# Autodesk Inventor assembly: driveFrameV2
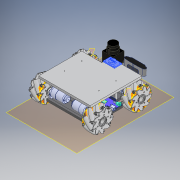
[picture p0: Inventor's stored thumbnail of the model, 180x180]
Saved by Autodesk Inventor 2017 (Build 210142000, 142)
## iProperties
Created: 2017-03-10
Part Number: driveFrameV2
Document SubType Name: Assembly
Designer: Naga
Author: Naga
## Documents named in this file (15)
- E:\GDrive\IEEE CS\SoutheastCon2017\Cad\Chassis\driveFrameV2.iam
- E:\GDrive\IEEE CS\SoutheastCon2017\Cad\Chassis\BottomPlateV2.ipt
- E:\GDrive\IEEE CS\SoutheastCon2017\Cad\Motors\37DEncoderAlBlock.iam
- E:\GDrive\IEEE CS\SoutheastCon2017\Cad\Chassis\TopPlateV1.ipt
- E:\GDrive\IEEE CS\SoutheastCon2017\Cad\Chassis\postSpacer.ipt
- E:\GDrive\IEEE CS\SoutheastCon2017\Cad\tilt\step\tiltservomount_std.iam
- E:\GDrive\IEEE CS\SoutheastCon2017\Cad\tilt\TiltMountShort.iam
- E:\GDrive\IEEE CS\SoutheastCon2017\Cad\pan\base.ipt
- E:\GDrive\IEEE CS\SoutheastCon2017\Cad\Motors\100mm Aluminum Mecanum wheels.iam
- E:\GDrive\IEEE CS\SoutheastCon2017\Cad\Electronics\Arduino Mega 2560.ipt
- E:\GDrive\IEEE CS\SoutheastCon2017\Cad\Electronics\RaspberryPi2 STEP214.iam
- E:\GDrive\IEEE CS\SoutheastCon2017\Cad\Electronics\kangarooSaberTooth.iam
- E:\GDrive\IEEE CS\SoutheastCon2017\Cad\Electronics\Lidar.ipt
- E:\GDrive\IEEE CS\SoutheastCon2017\Cad\Electronics\camera\LogitechC920Montaj.ipt
- E:\GDrive\IEEE CS\SoutheastCon2017\Cad\Motors\MG995_Servo.iam
## Components (24 placed, 14 different names)
1. BottomPlateV2:1 — Mate:3, Mate:4, Mate:5, Mate:6, Mate:7, Mate:8, Mate:9, Mate:16, Mate:20, Mate:21, Mate:22, Mate:23, Mate:24, Mate:25, Mate:26, Mate:50, Mate:51, Mate:52, Mate:53, Flush:26, Flush:27, Flush:29, Flush:30, Mate:56, Flush:33, Flush:38
2. 37DEncoderAlBlock:1 [sub-assembly] — Flush:2, Flush:3, Mate:5, Flush:4, Mate:6, Mate:48, Mate:49
3. 37DEncoderAlBlock:2 [sub-assembly] — Flush:1, Flush:5, Mate:9, Mate:44, Mate:46
4. 37DEncoderAlBlock:3 [sub-assembly] — Flush:3, Flush:5, Mate:8, Mate:45, Mate:47
5. 37DEncoderAlBlock:4 [sub-assembly] — Flush:1, Flush:2, Flush:4, Mate:7, Mate:42, Mate:43
6. TopPlateV1:1 — Mate:20, Mate:21, Mate:27, Mate:35, Flush:21, Mate:62
7. postSpacer:1 — Mate:24, Flush:12
8. postSpacer:2 — Mate:22, Flush:13, Flush:14, Mate:27
9. postSpacer:3 — Mate:23, Mate:26, Flush:12, Flush:13
10. postSpacer:4 — Mate:25, Flush:14
11. TiltMountShort:2 [sub-assembly] — Mate:31, Mate:56, Mate:57, Flush:33, Mate:59, Flush:38
12. tiltservomount_std:2 [sub-assembly] — Mate:31, Mate:55, Flush:31, Flush:32, Mate:57, Mate:60, Mate:61
13. base:1 — Mate:35, Flush:21
14. 100mm Aluminum Mecanum wheels:1 [sub-assembly] — Mate:42, Mate:43
15. 100mm Aluminum Mecanum wheels:2 [sub-assembly] — Mate:44, Mate:46
16. 100mm Aluminum Mecanum wheels:3 [sub-assembly] — Mate:45, Mate:47
17. 100mm Aluminum Mecanum wheels:4 [sub-assembly] — Mate:48, Mate:49
18. Arduino Mega 2560:1 — Mate:53, Flush:26
19. RaspberryPi2 STEP214:1 [sub-assembly] — Mate:52, Flush:27
20. kangarooSaberTooth:1 [sub-assembly] — Mate:51, Flush:29, Mate:54
21. kangarooSaberTooth:2 [sub-assembly] — Mate:50, Flush:30, Mate:54
22. Lidar:1 — Mate:55, Flush:31, Flush:32
23. LogitechC920Montaj:1 — Mate:62
24. MG995_Servo:1 [sub-assembly] — Mate:59, Mate:60, Mate:61
## Relationships (56: Mate 38, Flush 18)
- Mate:3: BottomPlateV2:1
- Mate:4: BottomPlateV2:1
- Flush:1: 37DEncoderAlBlock:2 ↔ 37DEncoderAlBlock:4
- Flush:2: 37DEncoderAlBlock:1 ↔ 37DEncoderAlBlock:4
- Flush:3: 37DEncoderAlBlock:1 ↔ 37DEncoderAlBlock:3
- Mate:5: BottomPlateV2:1 ↔ 37DEncoderAlBlock:1
- Flush:4: 37DEncoderAlBlock:1 ↔ 37DEncoderAlBlock:4
- Flush:5: 37DEncoderAlBlock:2 ↔ 37DEncoderAlBlock:3
- Mate:6: BottomPlateV2:1 ↔ 37DEncoderAlBlock:1
- Mate:7: BottomPlateV2:1 ↔ 37DEncoderAlBlock:4
- Mate:8: BottomPlateV2:1 ↔ 37DEncoderAlBlock:3
- Mate:9: BottomPlateV2:1 ↔ 37DEncoderAlBlock:2
- Mate:16 (32.1469 mm): BottomPlateV2:1
- Flush:10 (63.5 mm)
- Mate:20: BottomPlateV2:1 ↔ TopPlateV1:1
- Mate:21: BottomPlateV2:1 ↔ TopPlateV1:1
- Mate:22: BottomPlateV2:1 ↔ postSpacer:2
- Mate:23: BottomPlateV2:1 ↔ postSpacer:3
- Mate:24: BottomPlateV2:1 ↔ postSpacer:1
- Mate:25: BottomPlateV2:1 ↔ postSpacer:4
- Mate:26: BottomPlateV2:1 ↔ postSpacer:3
- Flush:12: postSpacer:1 ↔ postSpacer:3
- Flush:13: postSpacer:2 ↔ postSpacer:3
- Flush:14: postSpacer:2 ↔ postSpacer:4
- Mate:27: TopPlateV1:1 ↔ postSpacer:2
- Mate:31: TiltMountShort:2 ↔ tiltservomount_std:2
- Mate:35: TopPlateV1:1 ↔ base:1
- Flush:21: TopPlateV1:1 ↔ base:1
- Mate:42: 37DEncoderAlBlock:4 ↔ 100mm Aluminum Mecanum wheels:1
- Mate:43: 37DEncoderAlBlock:4 ↔ 100mm Aluminum Mecanum wheels:1
- Mate:44: 37DEncoderAlBlock:2 ↔ 100mm Aluminum Mecanum wheels:2
- Mate:45: 37DEncoderAlBlock:3 ↔ 100mm Aluminum Mecanum wheels:3
- Mate:46: 37DEncoderAlBlock:2 ↔ 100mm Aluminum Mecanum wheels:2
- Mate:47: 37DEncoderAlBlock:3 ↔ 100mm Aluminum Mecanum wheels:3
- Mate:48: 37DEncoderAlBlock:1 ↔ 100mm Aluminum Mecanum wheels:4
- Mate:49: 37DEncoderAlBlock:1 ↔ 100mm Aluminum Mecanum wheels:4
- Mate:50: BottomPlateV2:1 ↔ kangarooSaberTooth:2
- Mate:51: BottomPlateV2:1 ↔ kangarooSaberTooth:1
- Mate:52: BottomPlateV2:1 ↔ RaspberryPi2 STEP214:1
- Mate:53: BottomPlateV2:1 ↔ Arduino Mega 2560:1
- Flush:26: BottomPlateV2:1 ↔ Arduino Mega 2560:1
- Flush:27: BottomPlateV2:1 ↔ RaspberryPi2 STEP214:1
- Flush:29 (-19.05 mm): BottomPlateV2:1 ↔ kangarooSaberTooth:1
- Flush:30 (19.05 mm): BottomPlateV2:1 ↔ kangarooSaberTooth:2
- Mate:54: kangarooSaberTooth:1 ↔ kangarooSaberTooth:2
- Mate:55: tiltservomount_std:2 ↔ Lidar:1
- Flush:31: tiltservomount_std:2 ↔ Lidar:1
- Flush:32: tiltservomount_std:2 ↔ Lidar:1
- Mate:56: BottomPlateV2:1 ↔ TiltMountShort:2
- Mate:57: TiltMountShort:2 ↔ tiltservomount_std:2
- Flush:33: BottomPlateV2:1 ↔ TiltMountShort:2
- Mate:59: TiltMountShort:2 ↔ MG995_Servo:1
- Mate:60: tiltservomount_std:2 ↔ MG995_Servo:1
- Mate:61: tiltservomount_std:2 ↔ MG995_Servo:1
- Flush:38: BottomPlateV2:1 ↔ TiltMountShort:2
- Mate:62: TopPlateV1:1 ↔ LogitechC920Montaj:1
